# Autodesk Inventor assembly: final
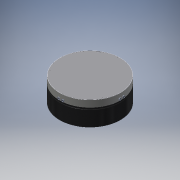
[picture p0: Inventor's stored thumbnail of the model, 180x180]
Saved by Autodesk Inventor 2019 (Build 230136000, 136)
## iProperties
Created: 2021-01-20
Part Number: final
Document SubType Name: Assembly
Designer: Admin
Author: Admin
## Documents named in this file (9)
- C:\Users\Admin\Documents\Inventor\Doan\final.iam
- C:\Users\Admin\Documents\Inventor\Doan\De_final.ipt
- C:\Users\Admin\Documents\Inventor\Doan\Banhxenew.iam
- C:\Users\Admin\Documents\Inventor\Doan\Than+CB.iam
- C:\Users\Admin\Documents\Inventor\Doan\then.ipt
- C:\Users\Admin\Documents\Inventor\Doan\Nap.ipt
- C:\Users\Admin\Documents\Inventor\Doan\trudong.ipt
- C:\Users\Admin\Documents\Inventor\Doan\napduoinew.ipt
- C:\Users\Admin\Documents\Inventor\Doan\trudong45mm.ipt
## Components (21 placed, 8 different names)
1. Than+CB:1 [sub-assembly] — Mate:4, Mate:5, Mate:6, Mate:7, Mate:8, Mate:9, Mate:10, Mate:13, Mate:14, Mate:17, Mate:18, Mate:20, Mate:29, Mate:30, Mate:31, Mate:32
2. then:2 — Mate:12
3. Nap:1 — Mate:13, Mate:14, Mate:20
4. De_final:1 — Mate:1, Mate:2, Mate:3, Mate:4, Mate:5, Mate:6, Mate:7, Mate:8, Mate:11, Mate:12, Mate:15, Mate:16, Mate:21, Mate:22, Mate:23, Mate:24, Mate:25, Mate:26, Mate:27, Mate:28
5. napduoinew:1 — Mate:17, Mate:18
6. trudong:5 — Mate:21, Mate:22
7. trudong:6 — Mate:23, Mate:24
8. trudong:7 — Mate:25, Mate:26
9. trudong:8 — Mate:27, Mate:28
10. trudong45mm:1 — Mate:29, Mate:30
11. trudong45mm:2 — Mate:31, Mate:32
12. Banhxenew:1 [sub-assembly] — Mate:1, Mate:2, Mate:3
13. Banhxenew:2 [sub-assembly]
14. Banhxenew:3 [sub-assembly]
15. then:1 — Mate:9, Mate:10, Mate:11
16. then:3
17. then:4
18. trudong:1 — Mate:15, Mate:16
19. trudong:2
20. trudong:3
21. trudong:4
## Component patterns: (3 elements, first: Banhxenew:1), (3 elements, first: then:1), (4 elements, first: trudong:1)
## Relationships (31: Mate 31)
- Mate:1: De_final:1 ↔ Banhxenew:1
- Mate:2: De_final:1 ↔ Banhxenew:1
- Mate:3: De_final:1 ↔ Banhxenew:1
- Mate:4: Than+CB:1 ↔ De_final:1
- Mate:5: Than+CB:1 ↔ De_final:1
- Mate:6: Than+CB:1 ↔ De_final:1
- Mate:7: Than+CB:1 ↔ De_final:1
- Mate:8: Than+CB:1 ↔ De_final:1
- Mate:9: Than+CB:1 ↔ then:1
- Mate:10: Than+CB:1 ↔ then:1
- Mate:11: De_final:1 ↔ then:1
- Mate:12: then:2 ↔ De_final:1
- Mate:13: Than+CB:1 ↔ Nap:1
- Mate:14: Than+CB:1 ↔ Nap:1
- Mate:15: De_final:1 ↔ trudong:1
- Mate:16: De_final:1 ↔ trudong:1
- Mate:17: Than+CB:1 ↔ napduoinew:1
- Mate:18: Than+CB:1 ↔ napduoinew:1
- Mate:20: Than+CB:1 ↔ Nap:1
- Mate:21: De_final:1 ↔ trudong:5
- Mate:22: De_final:1 ↔ trudong:5
- Mate:23: De_final:1 ↔ trudong:6
- Mate:24: De_final:1 ↔ trudong:6
- Mate:25: De_final:1 ↔ trudong:7
- Mate:26: De_final:1 ↔ trudong:7
- Mate:27: De_final:1 ↔ trudong:8
- Mate:28: De_final:1 ↔ trudong:8
- Mate:29: Than+CB:1 ↔ trudong45mm:1
- Mate:30: Than+CB:1 ↔ trudong45mm:1
- Mate:31: Than+CB:1 ↔ trudong45mm:2
- Mate:32: Than+CB:1 ↔ trudong45mm:2
